# Autodesk Inventor assembly: Cage
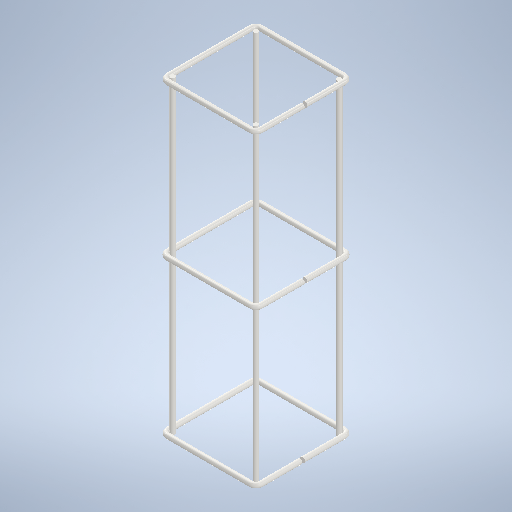
[picture p0: Inventor's stored thumbnail of the model, 512x512]
Saved by Autodesk Inventor 2025.1 (Build 291241020, 241B)
## iProperties
Created: 2024-09-07
Part Number: Cage
Document SubType Name: Assembly
Designer: Tom
Author: Tom
## Documents named in this file (3)
- C:\Users\Tom\Documents\Inventor\Mobility\Additional_Building\Cage.iam
- C:\Users\Tom\Documents\Inventor\Mobility\Additional_Building\Ring_Of_Rebar.ipt
- C:\Users\Tom\Documents\Inventor\Mobility\Additional_Building\Rebar_With_Length_Of_31.56275_Inches.ipt
## Components (7 placed, 2 different names)
1. Ring_Of_Rebar:1 — Flush:1, Flush:2, Flush:3, Tangent:1, Tangent:2, Tangent:3, Tangent:4, Tangent:5, Tangent:6, Tangent:7, Tangent:8, Tangent:9
2. Rebar_With_Length_Of_31.56275_Inches:1 — Mate:4, Tangent:8, Tangent:9, Tangent:10, Tangent:11, Mate:6, Tangent:18, Tangent:19
3. Rebar_With_Length_Of_31.56275_Inches:2 — Mate:3, Tangent:6, Tangent:7, Tangent:12, Tangent:13, Tangent:20, Tangent:21
4. Rebar_With_Length_Of_31.56275_Inches:3 — Mate:2, Tangent:4, Tangent:5, Tangent:14, Tangent:15, Tangent:22, Tangent:23
5. Rebar_With_Length_Of_31.56275_Inches:4 — Mate:1, Tangent:1, Tangent:2, Tangent:3, Tangent:16, Tangent:17, Tangent:24, Tangent:25
6. Ring_Of_Rebar:2 — Mate:5, Tangent:10, Tangent:11, Tangent:12, Tangent:13, Tangent:14, Tangent:15, Tangent:16, Tangent:17
7. Ring_Of_Rebar:3 — Mate:6, Tangent:18, Tangent:19, Tangent:20, Tangent:21, Tangent:22, Tangent:23, Tangent:24, Tangent:25
## Relationships (34: Tangent 25, Mate 6, Flush 3)
- Flush:1: Ring_Of_Rebar:1
- Flush:2: Ring_Of_Rebar:1
- Flush:3: Ring_Of_Rebar:1
- Mate:1 (-6.35 mm): Rebar_With_Length_Of_31.56275_Inches:4
- Tangent:1: Ring_Of_Rebar:1 ↔ Rebar_With_Length_Of_31.56275_Inches:4
- Tangent:2: Ring_Of_Rebar:1 ↔ Rebar_With_Length_Of_31.56275_Inches:4
- Tangent:3: Ring_Of_Rebar:1 ↔ Rebar_With_Length_Of_31.56275_Inches:4
- Mate:2 (-6.35 mm): Rebar_With_Length_Of_31.56275_Inches:3
- Tangent:4: Ring_Of_Rebar:1 ↔ Rebar_With_Length_Of_31.56275_Inches:3
- Tangent:5: Ring_Of_Rebar:1 ↔ Rebar_With_Length_Of_31.56275_Inches:3
- Mate:3: Rebar_With_Length_Of_31.56275_Inches:2
- Tangent:6: Ring_Of_Rebar:1 ↔ Rebar_With_Length_Of_31.56275_Inches:2
- Tangent:7: Ring_Of_Rebar:1 ↔ Rebar_With_Length_Of_31.56275_Inches:2
- Mate:4: Rebar_With_Length_Of_31.56275_Inches:1
- Tangent:8: Ring_Of_Rebar:1 ↔ Rebar_With_Length_Of_31.56275_Inches:1
- Tangent:9: Ring_Of_Rebar:1 ↔ Rebar_With_Length_Of_31.56275_Inches:1
- Mate:5 (400.8469 mm): Ring_Of_Rebar:2
- Tangent:10: Rebar_With_Length_Of_31.56275_Inches:1 ↔ Ring_Of_Rebar:2
- Tangent:11: Rebar_With_Length_Of_31.56275_Inches:1 ↔ Ring_Of_Rebar:2
- Tangent:12: Rebar_With_Length_Of_31.56275_Inches:2 ↔ Ring_Of_Rebar:2
- Tangent:13: Rebar_With_Length_Of_31.56275_Inches:2 ↔ Ring_Of_Rebar:2
- Tangent:14: Rebar_With_Length_Of_31.56275_Inches:3 ↔ Ring_Of_Rebar:2
- Tangent:15: Rebar_With_Length_Of_31.56275_Inches:3 ↔ Ring_Of_Rebar:2
- Tangent:16: Rebar_With_Length_Of_31.56275_Inches:4 ↔ Ring_Of_Rebar:2
- Tangent:17: Rebar_With_Length_Of_31.56275_Inches:4 ↔ Ring_Of_Rebar:2
- Mate:6 (-6.35 mm): Rebar_With_Length_Of_31.56275_Inches:1 ↔ Ring_Of_Rebar:3
- Tangent:18: Rebar_With_Length_Of_31.56275_Inches:1 ↔ Ring_Of_Rebar:3
- Tangent:19: Rebar_With_Length_Of_31.56275_Inches:1 ↔ Ring_Of_Rebar:3
- Tangent:20: Rebar_With_Length_Of_31.56275_Inches:2 ↔ Ring_Of_Rebar:3
- Tangent:21: Rebar_With_Length_Of_31.56275_Inches:2 ↔ Ring_Of_Rebar:3
- Tangent:22: Rebar_With_Length_Of_31.56275_Inches:3 ↔ Ring_Of_Rebar:3
- Tangent:23: Rebar_With_Length_Of_31.56275_Inches:3 ↔ Ring_Of_Rebar:3
- Tangent:24: Rebar_With_Length_Of_31.56275_Inches:4 ↔ Ring_Of_Rebar:3
- Tangent:25: Rebar_With_Length_Of_31.56275_Inches:4 ↔ Ring_Of_Rebar:3
